# Autodesk Inventor assembly: skellett
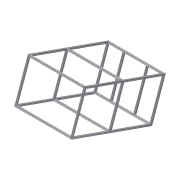
[picture p0: Inventor's stored thumbnail of the model, 180x180]
Saved by Autodesk Inventor 2014 SP1 (Build 180222100, 222)
## iProperties
Created: 2015-02-04
Part Number: skellett
Document SubType Name: Assembly
Designer: Simen
Author: Simen
## Documents named in this file (5)
- C:\Users\Simen\Documents\git\Eit\skjellet\skellett.iam
- C:\Users\Simen\Documents\git\Eit\skjellet\KHFS5_2020_1000.ipt
- C:\Users\Simen\Documents\git\Eit\skjellet\KHFS5_2020_500.ipt
- C:\Users\Simen\Documents\git\Eit\skjellet\KHFS5_2020_660.ipt
- C:\Users\Simen\Documents\git\Eit\skjellet\KHFS5_2020_460.ipt
## Components (18 placed, 1 different names)
1. KHFS5-2020-4000:6 — Mate:14, Flush:16, Flush:17, Flush:22, Flush:23, Mate:19
2. KHFS5-2020-4000:11
3. KHFS5-2020-4000:7 — Flush:20, Flush:21, Mate:18, Flush:22, Flush:23, Mate:19, Mate:20, Mate:21, Flush:28, Flush:29, Flush:30, Flush:31
4. KHFS5-2020-4000:8 — Flush:20, Flush:21, Mate:18, Mate:32
5. KHFS5-2020-4000:10
6. KHFS5-2020-4000:9 — Mate:14, Flush:16, Flush:17, Mate:22, Mate:23, Flush:24, Flush:25, Flush:26, Flush:27
7. KHFS5-2020-4000:12 — Mate:23, Flush:26, Flush:27, Mate:31, Flush:43
8. KHFS5-2020-4000:13 — Mate:22, Flush:24, Flush:25
9. KHFS5-2020-4000:19
10. KHFS5-2020-4000:14 — Mate:20, Flush:30, Flush:31, Flush:40, Mate:29
11. KHFS5-2020-4000:15 — Mate:21, Flush:28, Flush:29, Flush:41, Mate:28, Mate:30, Flush:42
12. KHFS5-2020-4000:16
13. KHFS5-2020-4000:17
14. KHFS5-2020-4000:18
15. KHFS5-2020-4000:20 — Flush:40, Mate:29, Flush:46, Mate:32
16. KHFS5-2020-4000:21 — Flush:41, Mate:28, Flush:44, Flush:45
17. KHFS5-2020-4000:22 — Mate:30, Flush:42, Flush:45, Flush:46
18. KHFS5-2020-4000:23 — Mate:31, Flush:43, Flush:44
## Relationships (49: Flush 31, Mate 18)
- Mate:14: KHFS5-2020-4000:6 ↔ KHFS5-2020-4000:9
- Flush:16: KHFS5-2020-4000:6 ↔ KHFS5-2020-4000:9
- Flush:17: KHFS5-2020-4000:6 ↔ KHFS5-2020-4000:9
- [Flush]: KHFS5-2020-4000:6 ↔ KHFS5-2020-4000:10
- [Mate]: KHFS5-2020-4000:6 ↔ KHFS5-2020-4000:10
- [Flush]: KHFS5-2020-4000:11 ↔ KHFS5-2020-4000:8
- [Mate]: KHFS5-2020-4000:11 ↔ KHFS5-2020-4000:8
- Flush:20: KHFS5-2020-4000:7 ↔ KHFS5-2020-4000:8
- Flush:21: KHFS5-2020-4000:7 ↔ KHFS5-2020-4000:8
- Mate:18: KHFS5-2020-4000:7 ↔ KHFS5-2020-4000:8
- Flush:22: KHFS5-2020-4000:6 ↔ KHFS5-2020-4000:7
- Flush:23: KHFS5-2020-4000:6 ↔ KHFS5-2020-4000:7
- Mate:19: KHFS5-2020-4000:6 ↔ KHFS5-2020-4000:7
- Mate:20: KHFS5-2020-4000:7 ↔ KHFS5-2020-4000:14
- Mate:21: KHFS5-2020-4000:7 ↔ KHFS5-2020-4000:15
- Mate:22: KHFS5-2020-4000:9 ↔ KHFS5-2020-4000:13
- Mate:23: KHFS5-2020-4000:9 ↔ KHFS5-2020-4000:12
- Flush:24: KHFS5-2020-4000:9 ↔ KHFS5-2020-4000:13
- Flush:25: KHFS5-2020-4000:9 ↔ KHFS5-2020-4000:13
- Flush:26: KHFS5-2020-4000:9 ↔ KHFS5-2020-4000:12
- Flush:27: KHFS5-2020-4000:9 ↔ KHFS5-2020-4000:12
- Flush:28: KHFS5-2020-4000:7 ↔ KHFS5-2020-4000:15
- Flush:29: KHFS5-2020-4000:7 ↔ KHFS5-2020-4000:15
- Flush:30: KHFS5-2020-4000:7 ↔ KHFS5-2020-4000:14
- Flush:31: KHFS5-2020-4000:7 ↔ KHFS5-2020-4000:14
- [Mate]: KHFS5-2020-4000:16 ↔ KHFS5-2020-4000:18
- [Flush]: KHFS5-2020-4000:16 ↔ KHFS5-2020-4000:18
- [Flush]: KHFS5-2020-4000:16 ↔ KHFS5-2020-4000:18
- [Flush]: KHFS5-2020-4000:17 ↔ KHFS5-2020-4000:18
- [Mate]: KHFS5-2020-4000:17 ↔ KHFS5-2020-4000:18
- [Flush]: KHFS5-2020-4000:17 ↔ KHFS5-2020-4000:18
- [Flush]: KHFS5-2020-4000:13 ↔ KHFS5-2020-4000:18
- [Mate]: KHFS5-2020-4000:13 ↔ KHFS5-2020-4000:18
- [Flush]: KHFS5-2020-4000:19 ↔ KHFS5-2020-4000:16
- [Flush]: KHFS5-2020-4000:19 ↔ KHFS5-2020-4000:16
- [Mate]: KHFS5-2020-4000:19 ↔ KHFS5-2020-4000:17
- [Flush]: KHFS5-2020-4000:13 ↔ KHFS5-2020-4000:19
- Flush:40: KHFS5-2020-4000:14 ↔ KHFS5-2020-4000:20
- Flush:41: KHFS5-2020-4000:15 ↔ KHFS5-2020-4000:21
- Mate:28: KHFS5-2020-4000:15 ↔ KHFS5-2020-4000:21
- Mate:29: KHFS5-2020-4000:14 ↔ KHFS5-2020-4000:20
- Mate:30: KHFS5-2020-4000:15 ↔ KHFS5-2020-4000:22
- Flush:42: KHFS5-2020-4000:15 ↔ KHFS5-2020-4000:22
- Mate:31: KHFS5-2020-4000:12 ↔ KHFS5-2020-4000:23
- Flush:43: KHFS5-2020-4000:12 ↔ KHFS5-2020-4000:23
- Flush:44: KHFS5-2020-4000:21 ↔ KHFS5-2020-4000:23
- Flush:45: KHFS5-2020-4000:21 ↔ KHFS5-2020-4000:22
- Flush:46: KHFS5-2020-4000:20 ↔ KHFS5-2020-4000:22
- Mate:32 (510 mm): KHFS5-2020-4000:8 ↔ KHFS5-2020-4000:20
